# Autodesk Inventor assembly: RForearm+rotation
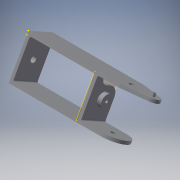
[picture p0: Inventor's stored thumbnail of the model, 180x180]
Saved by Autodesk Inventor 2018 (Build 220112000, 112)
## iProperties
Created: 2018-02-08
Part Number: RForearm+rotation
Material: Générique
Document SubType Name: Assembly
Designer: Thomas
Author: Thomas
## Documents named in this file (3)
- D:\Users\Thomas\Desktop\Projet robot augmenté\robotConcept\Right forearm\RForearm+rotation.iam
- D:\Users\Thomas\Desktop\Projet robot augmenté\robotConcept\Right forearm\Right forearm.ipt
- D:\Users\Thomas\Desktop\Projet robot augmenté\robotConcept\Right forearm\Forearm rotation.ipt
## Components (2 placed, 2 different names)
1. Right forearm:1 — Placage:1, Cylindrique:1
2. Forearm rotation:1 — Placage:1, Cylindrique:1
## Relationships (2: Mate 1, CylindricalJoint 1)
- Placage:1 [Mate]: Right forearm:1 ↔ Forearm rotation:1
- Cylindrique:1: Right forearm:1 ↔ Forearm rotation:1
